# Autodesk Inventor assembly: Stepper
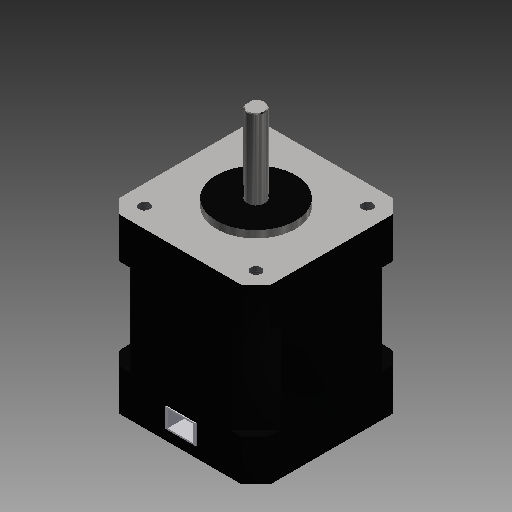
[picture p0: Inventor's stored thumbnail of the model, 512x512]
Saved by Autodesk Inventor 2018 (Build 220112000, 112)
## iProperties
Created: 2018-03-28
Part Number: Stepper
Document SubType Name: Assembly
Designer: Ajith Thomas
Author: Ajith Thomas
## Documents named in this file (4)
- C:\Users\Ajith Thomas\Dropbox\Gas_Sensing_Robot\FumeBot-Design\Stepper Motor\Stepper.iam
- C:\Users\Ajith Thomas\Dropbox\Gas_Sensing_Robot\FumeBot-Design\Stepper Motor\Stepper Motor.ipt
- C:\Users\Ajith Thomas\Dropbox\Gas_Sensing_Robot\FumeBot-Design\Stepper Motor\Stepper Shaft.ipt
- C:\Users\Ajith Thomas\Documents\Inventor\Content Center Files\R2018\en-US\ISO 7046-1 Z(1)\ISO 7046-1 - M3 x 4 - 4.8 - Z - ISO.ipt
## Components (6 placed, 3 different names)
1. Stepper Motor:1 — Insert:1, Insert:2, Insert:3, Insert:4, Insert:5, Stepper Drive
2. Stepper Shaft:1 — Insert:1, Stepper Drive
3. ISO 7046-1 Z M3 x 4 - 4.8 - Z:1 — Insert:2
4. ISO 7046-1 Z M3 x 4 - 4.8 - Z:2 — Insert:3
5. ISO 7046-1 Z M3 x 4 - 4.8 - Z:3 — Insert:4
6. ISO 7046-1 Z M3 x 4 - 4.8 - Z:4 — Insert:5
## Relationships (6: Insert 5, Angle 1)
- Insert:1: Stepper Motor:1 ↔ Stepper Shaft:1
- Insert:2: Stepper Motor:1 ↔ ISO 7046-1 Z M3 x 4 - 4.8 - Z:1
- Insert:3: Stepper Motor:1 ↔ ISO 7046-1 Z M3 x 4 - 4.8 - Z:2
- Insert:4: Stepper Motor:1 ↔ ISO 7046-1 Z M3 x 4 - 4.8 - Z:3
- Insert:5: Stepper Motor:1 ↔ ISO 7046-1 Z M3 x 4 - 4.8 - Z:4
- Stepper Drive [Angle] (0 deg): Stepper Motor:1 ↔ Stepper Shaft:1
